# Autodesk Inventor assembly: Mx64_with_horn_and_bearing_MIR1
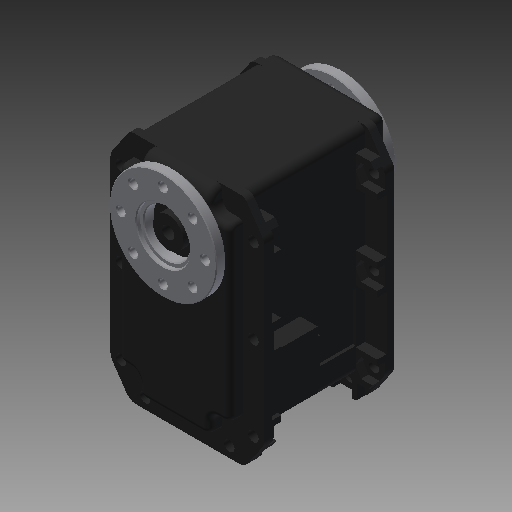
[picture p0: Inventor's stored thumbnail of the model, 512x512]
Saved by Autodesk Inventor 2019 (Build 230136000, 136)
## iProperties
Created: 2014-04-23
Part Number: Mx64_with_horn_and_bearing_MIR1
Document SubType Name: Assembly
Designer: 4wieser
Mass: 73.2688 g
Surface Area: 173.862 cm^2
Volume: 73.2688 cm^3
Density: 1 g/cm^3
Author: BitBots
## Documents named in this file (4)
- Z:\Nico_N\NICO-CAD-master\NICO_CAD_master\motors\Mx64\Mx64_with_horn_and_bearing_MIR1.iam
- Z:\Nico_N\NICO-CAD-master\NICO_CAD_master\motors\Mx64\MX-64T_MIR2.ipt
- Z:\Nico_N\NICO-CAD-master\NICO_CAD_master\motors\HN05-N101_(mx64)\HN05-N101_MIR2.ipt
- Z:\Nico_N\NICO-CAD-master\NICO_CAD_master\motors\HN05-i1_(mx64_bearing)\HN05-i1_MIR2.ipt
## Components (3 placed, 3 different names)
1. MX-64T_MIR2:1 — Rotational:3, Rotational:4
2. HN05-N101_MIR2:1 — Rotational:3
3. HN05-i1_MIR2:1 — Rotational:4
## Relationships (2: RevoluteJoint 2)
- Rotational:3 [RevoluteJoint]: MX-64T_MIR2:1 ↔ HN05-N101_MIR2:1
- Rotational:4 [RevoluteJoint]: MX-64T_MIR2:1 ↔ HN05-i1_MIR2:1
